# Autodesk Inventor assembly: Swerve-Drivetrain-2
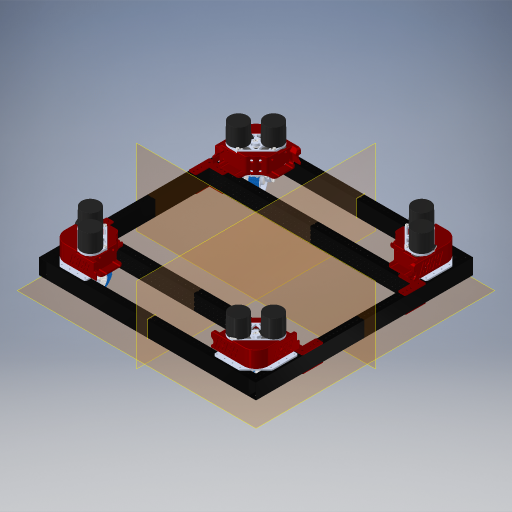
[picture p0: Inventor's stored thumbnail of the model, 512x512]
Saved by Autodesk Inventor 2024.2 (Build 282272000, 272)
## iProperties
Created: 2024-01-06
Part Number: Swerve-Drivetrain-2
Document SubType Name: Assembly
Designer: rohan
Author: rohan
## Documents named in this file (6)
- C:\Users\rohan\OneDrive - Hillsborough County Public Schools\Robotics\FIRST-Robotics-Competition\Crescendo\Minotaur-Crescendo-Robot\Swerve-Drivetrain.iam
- C:\Users\rohan\OneDrive - Hillsborough County Public Schools\Robotics\FIRST-Robotics-Competition\Crescendo\Minotaur-Crescendo-Robot\Motion\Swerve-Modules\MK3-Swerve-Module-Neos.iam
- C:\Users\rohan\OneDrive - Hillsborough County Public Schools\Robotics\FIRST-Robotics-Competition\Crescendo\Minotaur-Crescendo-Robot\Structure\MAXTube\2024-100-002-Front-Back-Extrusions.ipt
- C:\Users\rohan\OneDrive - Hillsborough County Public Schools\Robotics\FIRST-Robotics-Competition\Crescendo\Minotaur-Crescendo-Robot\Structure\MAXTube\2024-100-001-Left-Right-Extrusions.ipt
- C:\Users\rohan\OneDrive - Hillsborough County Public Schools\Robotics\FIRST-Robotics-Competition\Crescendo\Minotaur-Crescendo-Robot\Structure\MAXTube\2024-100-003-Middle-Extrusions.ipt
- C:\Users\rohan\OneDrive - Hillsborough County Public Schools\Robotics\FIRST-Robotics-Competition\Crescendo\Minotaur-Crescendo-Robot\Structure\Gussets\THRIFYBOT-L-Gusset.ipt
## Components (18 placed, 5 different names)
1. MK3-Swerve-Module-Neos:1 [sub-assembly] — Mate:75, Mate:80, Mate:81
2. MK3-Swerve-Module-Neos:2 [sub-assembly] — Mate:74, Mate:82, Mate:83
3. MK3-Swerve-Module-Neos:3 [sub-assembly] — Mate:73, Mate:76, Mate:77
4. MK3-Swerve-Module-Neos:4 [sub-assembly] — Mate:72, Mate:78, Mate:79
5. 2024-100-001-Left-Right-Extrusions:1 — Mate:69, Flush:1, Flush:2, Mate:70, Flush:3, Flush:4, Mate:73, Mate:76, Mate:82
6. 2024-100-001-Left-Right-Extrusions:2 — Mate:71, Flush:5, Flush:6, Mate:79, Mate:81
7. 2024-100-002-Front-Back-Extrusions:1 — Mate:70, Flush:3, Flush:4, Mate:72, Mate:77, Mate:78, Mate:84, Mate:85, Mate:94, Flush:22, Mate:95, Flush:23
8. 2024-100-002-Front-Back-Extrusions:2 — Mate:69, Flush:1, Flush:2, Mate:71, Flush:5, Flush:6, Mate:74, Mate:75, Mate:80, Mate:83, Flush:7, Flush:8, Flush:18, Mate:91, Mate:92, Flush:20, Mate:93
9. 2024-100-003-Middle-Extrusions:1 — Mate:85, Flush:7, Mate:90, Flush:17, Flush:21
10. 2024-100-003-Middle-Extrusions:2 — Mate:84, Flush:8, Flush:19, Flush:24
11. THRIFYBOT-L-Gusset:1 — Flush:15, Flush:16, Mate:89, Mate:90, Flush:17, Flush:18, Mate:91
12. THRIFYBOT-L-Gusset:2 — Flush:15, Flush:16, Mate:89
13. THRIFYBOT-L-Gusset:3 — Flush:13, Flush:14, Mate:88, Mate:95, Flush:23, Flush:24
14. THRIFYBOT-L-Gusset:4 — Flush:13, Flush:14, Mate:88
15. THRIFYBOT-L-Gusset:5 — Flush:11, Flush:12, Mate:87, Mate:94, Flush:21, Flush:22
16. THRIFYBOT-L-Gusset:6 — Flush:11, Flush:12, Mate:87
17. THRIFYBOT-L-Gusset:7 — Flush:9, Flush:10, Mate:86
18. THRIFYBOT-L-Gusset:8 — Flush:9, Flush:10, Mate:86, Mate:92, Flush:19, Flush:20, Mate:93
## Relationships (51: Mate 27, Flush 24)
- Mate:69: 2024-100-001-Left-Right-Extrusions:1 ↔ 2024-100-002-Front-Back-Extrusions:2
- Flush:1: 2024-100-001-Left-Right-Extrusions:1 ↔ 2024-100-002-Front-Back-Extrusions:2
- Flush:2: 2024-100-001-Left-Right-Extrusions:1 ↔ 2024-100-002-Front-Back-Extrusions:2
- Mate:70: 2024-100-001-Left-Right-Extrusions:1 ↔ 2024-100-002-Front-Back-Extrusions:1
- Flush:3: 2024-100-001-Left-Right-Extrusions:1 ↔ 2024-100-002-Front-Back-Extrusions:1
- Flush:4: 2024-100-001-Left-Right-Extrusions:1 ↔ 2024-100-002-Front-Back-Extrusions:1
- Mate:71: 2024-100-001-Left-Right-Extrusions:2 ↔ 2024-100-002-Front-Back-Extrusions:2
- Flush:5: 2024-100-001-Left-Right-Extrusions:2 ↔ 2024-100-002-Front-Back-Extrusions:2
- Flush:6: 2024-100-001-Left-Right-Extrusions:2 ↔ 2024-100-002-Front-Back-Extrusions:2
- Mate:72: MK3-Swerve-Module-Neos:4 ↔ 2024-100-002-Front-Back-Extrusions:1
- Mate:73: MK3-Swerve-Module-Neos:3 ↔ 2024-100-001-Left-Right-Extrusions:1
- Mate:74: MK3-Swerve-Module-Neos:2 ↔ 2024-100-002-Front-Back-Extrusions:2
- Mate:75: MK3-Swerve-Module-Neos:1 ↔ 2024-100-002-Front-Back-Extrusions:2
- Mate:76: MK3-Swerve-Module-Neos:3 ↔ 2024-100-001-Left-Right-Extrusions:1
- Mate:77: MK3-Swerve-Module-Neos:3 ↔ 2024-100-002-Front-Back-Extrusions:1
- Mate:78: MK3-Swerve-Module-Neos:4 ↔ 2024-100-002-Front-Back-Extrusions:1
- Mate:79: MK3-Swerve-Module-Neos:4 ↔ 2024-100-001-Left-Right-Extrusions:2
- Mate:80: MK3-Swerve-Module-Neos:1 ↔ 2024-100-002-Front-Back-Extrusions:2
- Mate:81: MK3-Swerve-Module-Neos:1 ↔ 2024-100-001-Left-Right-Extrusions:2
- Mate:82: MK3-Swerve-Module-Neos:2 ↔ 2024-100-001-Left-Right-Extrusions:1
- Mate:83: MK3-Swerve-Module-Neos:2 ↔ 2024-100-002-Front-Back-Extrusions:2
- Mate:84: 2024-100-002-Front-Back-Extrusions:1 ↔ 2024-100-003-Middle-Extrusions:2
- Mate:85: 2024-100-002-Front-Back-Extrusions:1 ↔ 2024-100-003-Middle-Extrusions:1
- Flush:7: 2024-100-002-Front-Back-Extrusions:2 ↔ 2024-100-003-Middle-Extrusions:1
- Flush:8: 2024-100-002-Front-Back-Extrusions:2 ↔ 2024-100-003-Middle-Extrusions:2
- Flush:9: THRIFYBOT-L-Gusset:7 ↔ THRIFYBOT-L-Gusset:8
- Flush:10: THRIFYBOT-L-Gusset:7 ↔ THRIFYBOT-L-Gusset:8
- Mate:86 (50.8 mm): THRIFYBOT-L-Gusset:7 ↔ THRIFYBOT-L-Gusset:8
- Flush:11: THRIFYBOT-L-Gusset:5 ↔ THRIFYBOT-L-Gusset:6
- Flush:12: THRIFYBOT-L-Gusset:5 ↔ THRIFYBOT-L-Gusset:6
- Mate:87 (50.8 mm): THRIFYBOT-L-Gusset:5 ↔ THRIFYBOT-L-Gusset:6
- Flush:13: THRIFYBOT-L-Gusset:3 ↔ THRIFYBOT-L-Gusset:4
- Flush:14: THRIFYBOT-L-Gusset:3 ↔ THRIFYBOT-L-Gusset:4
- Mate:88 (50.8 mm): THRIFYBOT-L-Gusset:3 ↔ THRIFYBOT-L-Gusset:4
- Flush:15: THRIFYBOT-L-Gusset:1 ↔ THRIFYBOT-L-Gusset:2
- Flush:16: THRIFYBOT-L-Gusset:1 ↔ THRIFYBOT-L-Gusset:2
- Mate:89 (50.8 mm): THRIFYBOT-L-Gusset:1 ↔ THRIFYBOT-L-Gusset:2
- Mate:90: 2024-100-003-Middle-Extrusions:1 ↔ THRIFYBOT-L-Gusset:1
- Flush:17: 2024-100-003-Middle-Extrusions:1 ↔ THRIFYBOT-L-Gusset:1
- Flush:18: 2024-100-002-Front-Back-Extrusions:2 ↔ THRIFYBOT-L-Gusset:1
- Mate:91: 2024-100-002-Front-Back-Extrusions:2 ↔ THRIFYBOT-L-Gusset:1
- Mate:92: 2024-100-002-Front-Back-Extrusions:2 ↔ THRIFYBOT-L-Gusset:8
- Flush:19: 2024-100-003-Middle-Extrusions:2 ↔ THRIFYBOT-L-Gusset:8
- Flush:20: 2024-100-002-Front-Back-Extrusions:2 ↔ THRIFYBOT-L-Gusset:8
- Mate:93: 2024-100-002-Front-Back-Extrusions:2 ↔ THRIFYBOT-L-Gusset:8
- Mate:94: 2024-100-002-Front-Back-Extrusions:1 ↔ THRIFYBOT-L-Gusset:5
- Flush:21: 2024-100-003-Middle-Extrusions:1 ↔ THRIFYBOT-L-Gusset:5
- Flush:22: 2024-100-002-Front-Back-Extrusions:1 ↔ THRIFYBOT-L-Gusset:5
- Mate:95: 2024-100-002-Front-Back-Extrusions:1 ↔ THRIFYBOT-L-Gusset:3
- Flush:23: 2024-100-002-Front-Back-Extrusions:1 ↔ THRIFYBOT-L-Gusset:3
- Flush:24: 2024-100-003-Middle-Extrusions:2 ↔ THRIFYBOT-L-Gusset:3
